# Autodesk Inventor assembly: CycloidalGearBoxAssembly_Stage2
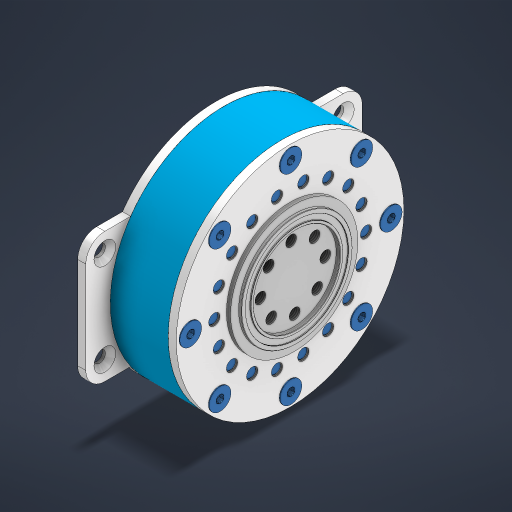
[picture p0: Inventor's stored thumbnail of the model, 512x512]
Saved by Autodesk Inventor 2024 (Build 280153000, 153)
## iProperties
Created: 2024-02-26
Part Number: CycloidalGearBoxAssembly_Stage2
Document SubType Name: Assembly
Designer: avsar
Author: avsar
## Documents named in this file (3)
- C:\Users\avsar\Documents\Inventor\RCR_Arm\Arm_V4\CycloidalGearBoxes\StageTwoGearBox\CycloidalGearBoxAssembly_Stage2.iam
- C:\Users\avsar\Documents\Inventor\RCR_Arm\Arm_V4\CycloidalGearBoxes\StageOneGearBox\CycloidalGearBoxAssemblyV2.iam
- C:\Users\avsar\Documents\Inventor\RCR_Arm\Arm_V4\CycloidalGearBoxes\StageOneGearBox\EccentricBearingShaft_8mmBore.ipt
## Components (2 placed, 2 different names)
1. CycloidalGearBoxAssemblyV2:1 [sub-assembly] — Flush:1, Mate:1, Mate:2
2. EccentricBearingShaft_8mmBore:1 — Flush:1, Mate:1, Mate:2
## Relationships (3: Mate 2, Flush 1)
- Flush:1: CycloidalGearBoxAssemblyV2:1 ↔ EccentricBearingShaft_8mmBore:1
- Mate:1: CycloidalGearBoxAssemblyV2:1 ↔ EccentricBearingShaft_8mmBore:1
- Mate:2: CycloidalGearBoxAssemblyV2:1 ↔ EccentricBearingShaft_8mmBore:1
